# Autodesk Inventor assembly: S4x2
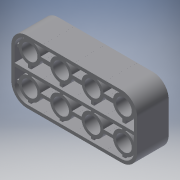
[picture p0: Inventor's stored thumbnail of the model, 180x180]
Saved by Autodesk Inventor 2019.3 (Build 233278000, 278)
## iProperties
Created: 2019-01-31
Part Number: S4x2
Document SubType Name: Assembly
Designer: Varga Daniel
Author: Varga Daniel
## Documents named in this file (4)
- C:\!_Dani\!_cloud\OneDrive\!_munka\Revolution\RevvyDemoKit\Structural parts\Beams\Straight Beams\S2+x2\S4x2.iam
- C:\!_Dani\!_cloud\OneDrive\!_munka\Revolution\RevvyDemoKit\Structural parts\Beams\beam_corner_part.ipt
- C:\!_Dani\!_cloud\OneDrive\!_munka\Revolution\RevvyDemoKit\Structural parts\Beams\beam_side_part.ipt
- C:\!_Dani\!_cloud\OneDrive\!_munka\Revolution\RevvyDemoKit\Structural parts\Beams\Straight Beams\S2+x2.iam
## Components (8 placed, 2 different names)
1. beam_corner_part:1 — Flush:1, Flush:2, Mate:1, Flush:7, Mate:4, Flush:8, Flush:9, Mate:5, Flush:10
2. beam_corner_part:2 — Flush:1, Flush:2, Mate:1
3. beam_corner_part:3 — Flush:5, Flush:6, Mate:3, Flush:7, Mate:4, Flush:10
4. beam_corner_part:4 — Flush:5, Flush:6, Mate:3
5. beam_side_part:1 — Mate:2, Flush:3, Flush:4, Flush:8, Flush:9, Mate:5
6. beam_side_part:2 — Mate:2, Flush:3, Flush:4
7. beam_side_part:3
8. beam_side_part:4
## Component patterns: (2 elements, first: beam_side_part:1 + beam_side_part:2)
## Relationships (15: Flush 10, Mate 5)
- Flush:1: beam_corner_part:1 ↔ beam_corner_part:2
- Flush:2: beam_corner_part:1 ↔ beam_corner_part:2
- Mate:1: beam_corner_part:1 ↔ beam_corner_part:2
- Mate:2: beam_side_part:1 ↔ beam_side_part:2
- Flush:3: beam_side_part:1 ↔ beam_side_part:2
- Flush:4: beam_side_part:1 ↔ beam_side_part:2
- Flush:5: beam_corner_part:3 ↔ beam_corner_part:4
- Flush:6: beam_corner_part:3 ↔ beam_corner_part:4
- Mate:3: beam_corner_part:3 ↔ beam_corner_part:4
- Flush:7: beam_corner_part:1 ↔ beam_corner_part:3
- Mate:4 (20 mm): beam_corner_part:1 ↔ beam_corner_part:3
- Flush:8: beam_corner_part:1 ↔ beam_side_part:1
- Flush:9: beam_corner_part:1 ↔ beam_side_part:1
- Mate:5: beam_corner_part:1 ↔ beam_side_part:1
- Flush:10: beam_corner_part:1 ↔ beam_corner_part:3
